# Autodesk Inventor assembly: CL7-200
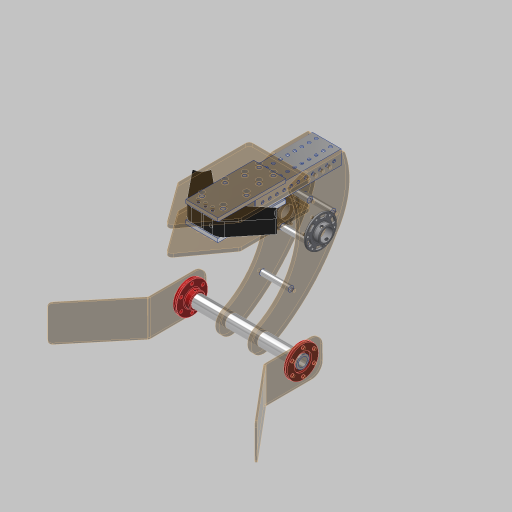
[picture p0: Inventor's stored thumbnail of the model, 512x512]
Saved by Autodesk Inventor 2023.5 (Build 275446000, 446)
## iProperties
Created: 2025-03-17
Part Number: CL7-200
Document SubType Name: Assembly
Designer: dlangdon
Mass: 1220.61 g
Surface Area: 3383.48 cm^2
Volume: 822.66 cm^3
Density: 1.48373 g/cm^3
Author: dlangdon
## Documents named in this file (13)
- C:\Users\slick\OneDrive\Desktop\2025-ReefScape---CAD\Climber\CL7\CL7-200.iam
- C:\Users\slick\OneDrive\Desktop\2025-ReefScape---CAD\Climber\CL7\CL7-005.ipt
- C:\Users\slick\OneDrive\Desktop\2025-ReefScape---CAD\Climber\CL7\CL7-004.ipt
- C:\Users\slick\OneDrive\Desktop\2025-ReefScape---CAD\Climber\CL7\CL7-005aa.ipt
- C:\Users\slick\OneDrive\Desktop\2025-ReefScape---CAD\Climber\CL7\CL7-006.ipt
- C:\Users\slick\OneDrive\Desktop\2025-ReefScape---CAD\Climber\CL7\CL7-008.ipt
- C:\Users\slick\OneDrive\Desktop\2025-ReefScape---CAD\Climber\CL7\CL7-009.ipt
- C:\Users\slick\OneDrive\Desktop\2025-ReefScape---CAD\Climber\CL7\CL-GB\CL7-GB-005.ipt
- C:\Users\slick\OneDrive\Desktop\2025-ReefScape---CAD\Climber\CL7\CL7-017.ipt
- C:\Users\slick\OneDrive\Desktop\2025-ReefScape---CAD\Climber\CL7\CL7-019.ipt
- C:\Users\slick\OneDrive\Desktop\2025-ReefScape---CAD\STEP files\CLIMBER LATCH SPACER.ipt
- C:\Users\slick\OneDrive\Desktop\2025-ReefScape---CAD\Climber\CL7\CL7-022.ipt
- C:\Users\slick\OneDrive\Desktop\2025-ReefScape---CAD\Climber\CL7\CL7-023.ipt
## Components (22 placed, 12 different names)
1. CL7-005:1 — Mate:4, Mate:5, Mate:6, Mate:7, Mate:8, Mate:9, Insert:1, Insert:2, Insert:13, Insert:14
2. CL7-004:1 — Mate:5, Flush:1, Symmetry:2, Flush:2, Insert:22
3. CL7-004:2 — Mate:4, Mate:6, Flush:1, Symmetry:2, Flush:2, Insert:21
4. CL7-005aa:1 — Mate:7, Mate:8, Mate:9, Insert:15, Insert:16
5. CL7-006:1 — Insert:1, Insert:2, Insert:3, Insert:4, Insert:5, Insert:6, Insert:7, Insert:8
6. CL7-008:1 — Insert:3, Insert:4, Symmetry:1, Insert:8, Insert:11, Insert:12, Insert:17, Insert:18, Insert:19, Insert:20
7. CL7-008:2 — Insert:5, Insert:6, Symmetry:1, Mate:10, Insert:7, Insert:9, Insert:10
8. CL7-009:1 — Mate:10, Mate:11, Mate:12, Mate:13, Flush:3, Flush:4
9. CL7-GB-005:1 — Insert:11, Insert:12
10. CL7-GB-005:2 — Insert:9, Insert:10
11. CL7-017:1 — Insert:13, Insert:14
12. CL7-017:2 — Insert:15, Insert:16
13. CL7-019:1 — Insert:17
14. CL7-019:2 — Insert:18
15. CL7-019:3 — Insert:19
16. CL7-019:4 — Insert:20
17. CLIMBER LATCH SPACER:1 — Insert:21
18. CLIMBER LATCH SPACER:2 — Insert:22
19. CL7-022:1 — Mate:12, Flush:4, Mate:15, Insert:25
20. CL7-022:2 — Mate:13, Flush:3, Mate:14, Insert:23, Insert:24
21. CL7-023:1 — Mate:14, Insert:23, Insert:24, Flush:5, Flush:6
22. CL7-023:2 — Mate:15, Flush:5, Flush:6, Insert:25
## Relationships (45: Insert 25, Mate 12, Flush 6, Symmetry 2)
- Mate:4: CL7-005:1 ↔ CL7-004:2
- Mate:5: CL7-005:1 ↔ CL7-004:1
- Mate:6 (0.7937 mm): CL7-005:1 ↔ CL7-004:2
- Flush:1: CL7-004:1 ↔ CL7-004:2
- Mate:7: CL7-005:1 ↔ CL7-005aa:1
- Mate:8: CL7-005:1 ↔ CL7-005aa:1
- Mate:9 (25.4 mm): CL7-005:1 ↔ CL7-005aa:1
- Insert:1: CL7-005:1 ↔ CL7-006:1
- Insert:2: CL7-005:1 ↔ CL7-006:1
- Insert:3: CL7-006:1 ↔ CL7-008:1
- Insert:4: CL7-006:1 ↔ CL7-008:1
- Insert:5: CL7-006:1 ↔ CL7-008:2
- Insert:6: CL7-006:1 ↔ CL7-008:2
- Symmetry:1: CL7-008:1 ↔ CL7-008:2
- Mate:10: CL7-008:2 ↔ CL7-009:1
- Mate:11: CL7-009:1
- Insert:7: CL7-006:1 ↔ CL7-008:2
- Insert:8: CL7-006:1 ↔ CL7-008:1
- Symmetry:2: CL7-004:1 ↔ CL7-004:2
- Flush:2: CL7-004:1 ↔ CL7-004:2
- Insert:9: CL7-008:2 ↔ CL7-GB-005:2
- Insert:10: CL7-008:2 ↔ CL7-GB-005:2
- Insert:11: CL7-008:1 ↔ CL7-GB-005:1
- Insert:12: CL7-008:1 ↔ CL7-GB-005:1
- Insert:13: CL7-005:1 ↔ CL7-017:1
- Insert:14: CL7-005:1 ↔ CL7-017:1
- Insert:15: CL7-005aa:1 ↔ CL7-017:2
- Insert:16: CL7-005aa:1 ↔ CL7-017:2
- Insert:17: CL7-008:1 ↔ CL7-019:1
- Insert:18: CL7-008:1 ↔ CL7-019:2
- Insert:19: CL7-008:1 ↔ CL7-019:3
- Insert:20: CL7-008:1 ↔ CL7-019:4
- Insert:21: CL7-004:2 ↔ CLIMBER LATCH SPACER:1
- Insert:22: CL7-004:1 ↔ CLIMBER LATCH SPACER:2
- Mate:12: CL7-009:1 ↔ CL7-022:1
- Mate:13: CL7-009:1 ↔ CL7-022:2
- Flush:3: CL7-009:1 ↔ CL7-022:2
- Flush:4: CL7-009:1 ↔ CL7-022:1
- Mate:14: CL7-022:2 ↔ CL7-023:1
- Insert:23: CL7-022:2 ↔ CL7-023:1
- Insert:24: CL7-022:2 ↔ CL7-023:1
- Mate:15: CL7-022:1 ↔ CL7-023:2
- Flush:5: CL7-023:1 ↔ CL7-023:2
- Flush:6: CL7-023:1 ↔ CL7-023:2
- Insert:25: CL7-022:1 ↔ CL7-023:2
